# Autodesk Inventor assembly: wheel_axle_MIR
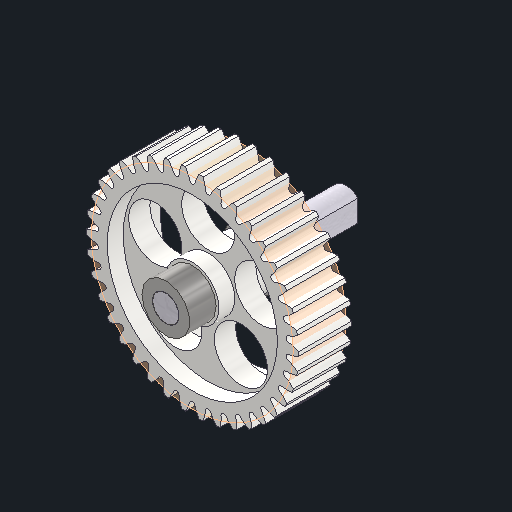
[picture p0: Inventor's stored thumbnail of the model, 512x512]
Saved by Autodesk Inventor 2023 (Build 270158000, 158)
## iProperties
Created: 2024-04-09
Part Number: wheel_axle_MIR
Document SubType Name: Assembly
Designer: szymo
Mass: 20.4365 g
Surface Area: 69.3563 cm^2
Volume: 6.5273 cm^3
Density: 3.13093 g/cm^3
Author: szymo
## Documents named in this file (5)
- C:\zRozne\roboilo\robots\codename wafel - australia\3d_parts\wheel_axle_MIR.iam
- C:\zRozne\roboilo\robots\codename wafel - australia\3d_parts\wal_kola_MIR.ipt
- C:\zRozne\roboilo\robots\codename wafel - australia\3d_parts\MegaSumo kola zebate 38_MIR.ipt
- C:\zRozne\roboilo\robots\codename wafel - australia\3d_parts\small_bearing_MIR.ipt
- C:\zRozne\roboilo\robots\codename wafel - australia\3d_parts\big_bearing_MIR.ipt
## Components (4 placed, 4 different names)
1. wal_kola_MIR:1 — Flush:1, Flush:2, Rotational:1
2. MegaSumo kola zebate 38_MIR:1 — Rotational:1
3. small_bearing_MIR:1 — Flush:1
4. big_bearing_MIR:1 — Flush:2
## Relationships (3: Mate 2, RevoluteJoint 1)
- Flush:1 [Mate]: wal_kola_MIR:1 ↔ small_bearing_MIR:1
- Flush:2 [Mate]: wal_kola_MIR:1 ↔ big_bearing_MIR:1
- Rotational:1 [RevoluteJoint]: wal_kola_MIR:1 ↔ MegaSumo kola zebate 38_MIR:1
